# Autodesk Inventor assembly: Montagem1
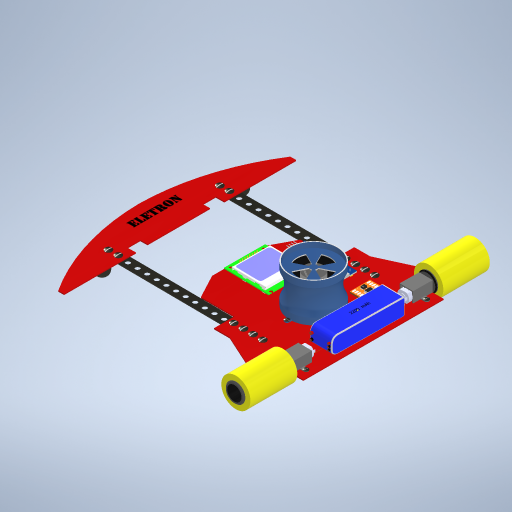
[picture p0: Inventor's stored thumbnail of the model, 512x512]
Saved by Autodesk Inventor 2023 (Build 270158000, 158)
## iProperties
Created: 2023-08-10
Part Number: Montagem1
Document SubType Name: Assembly
Designer: azeve
Author: azeve
## Documents named in this file (19)
- C:\Users\azeve\OneDrive\Área de Trabalho\seguidor_linha\Montagem1.iam
- C:\Users\azeve\OneDrive\Área de Trabalho\seguidor_linha\base_1.ipt
- C:\Users\azeve\OneDrive\Área de Trabalho\seguidor_linha\roda.ipt
- C:\Users\azeve\OneDrive\Área de Trabalho\cad_seguidor\Peças GrabCad\n20-motor-1.snapshot.1\N20 Motor.ipt
- C:\Users\azeve\OneDrive\Área de Trabalho\seguidor_linha\engate_motor.ipt
- C:\Users\azeve\OneDrive\Área de Trabalho\seguidor_linha\bateria.ipt
- C:\Users\azeve\OneDrive\Área de Trabalho\seguidor_linha\acoplamento_ventoinha1.ipt
- C:\Users\azeve\OneDrive\Área de Trabalho\seguidor_linha\aste2.ipt
- C:\Users\azeve\OneDrive\Área de Trabalho\seguidor_linha\sensor3.ipt
- C:\Users\azeve\OneDrive\Área de Trabalho\seguidor_linha\esfera.ipt
- C:\Users\azeve\OneDrive\Área de Trabalho\seguidor_linha\acoplamento_esfera.ipt
- C:\Users\azeve\OneDrive\Área de Trabalho\seguidor_linha\pneu.ipt
- C:\Users\azeve\OneDrive\Área de Trabalho\seguidor_linha\motor_ven.ipt
- C:\Users\azeve\OneDrive\Área de Trabalho\seguidor_linha\prafuso3.ipt
- C:\Users\azeve\OneDrive\Área de Trabalho\seguidor_linha\parafusos.ipt
- C:\Users\azeve\OneDrive\Área de Trabalho\seguidor_linha\helice.ipt
- C:\Users\azeve\OneDrive\Área de Trabalho\cad_seguidor\Peças GrabCad\nokia-5110-1.snapshot.1\Nokia 5110.ipt
- C:\Users\azeve\OneDrive\Área de Trabalho\cad_seguidor\Peças GrabCad\sparkfun-motor-driver-dual-tb6612fng-1a-1.snapshot.5\Motor Driver.ipt
- C:\Users\azeve\OneDrive\Área de Trabalho\cad_seguidor\Peças GrabCad\stm32f103c8t6-board-1.snapshot.2\stm32f103c8t6-board.ipt
## Components (43 placed, 18 different names)
1. base_1:1 — Coincidente:3, Coincidente:5, Coincidente:7, Coincidente:8, Coincidente:10, Coincidente:12, Alinhado:1, Inserir:20, Inserir:21, Inserir:22, Inserir:23, Inserir:24, Inserir:25, Inserir:26, Inserir:27, Coincidente:16, Coincidente:17
2. roda:1 — Inserir:4, Inserir:6
3. roda:2 — Inserir:3, Inserir:5
4. N20 Motor:1 — Coincidente:3, Coincidente:4, Inserir:4
5. N20 Motor:2 — Coincidente:1, Coincidente:2, Coincidente:5, Inserir:3
6. engate_motor:1 — Inserir:12, Inserir:13
7. engate_motor:2 — Inserir:14, Inserir:15
8. bateria:1
9. acoplamento_ventoinha1:1 — Inserir:7, Inserir:8, Inserir:9, Inserir:10, Inserir:11, Inserir:28
10. aste2:1 — Coincidente:8, Coincidente:11, Coincidente:12
11. aste2:2 — Coincidente:7, Coincidente:9, Coincidente:10
12. sensor3:1 — Coincidente:9, Coincidente:11, Coincidente:14, Coincidente:15, Inserir:16, Inserir:17, Inserir:18, Inserir:19
13. esfera:1 — Tangente:1
14. esfera:2 — Coincidente:13
15. acoplamento_esfera:1 — Tangente:1, Coincidente:15
16. acoplamento_esfera:2 — Coincidente:13, Coincidente:14
17. pneu:1 — Inserir:5
18. pneu:2 — Inserir:6
19. motor_ven:1 — Inserir:7
20. prafuso3:1 — Inserir:9
21. prafuso3:2 — Inserir:15
22. prafuso3:3 — Inserir:11
23. prafuso3:4 — Inserir:8
24. prafuso3:5 — Inserir:13
25. prafuso3:6 — Inserir:12
26. prafuso3:7 — Inserir:14
27. prafuso3:8 — Inserir:10
28. parafusos:1 — Inserir:20
29. parafusos:2 — Inserir:21
30. parafusos:3 — Inserir:22
31. parafusos:4 — Inserir:23
32. parafusos:5 — Inserir:24
33. parafusos:6 — Inserir:27
34. parafusos:7 — Inserir:25
35. parafusos:8 — Inserir:26
36. parafusos:9 — Inserir:18
37. parafusos:10 — Inserir:19
38. parafusos:11 — Inserir:16
39. parafusos:12 — Inserir:17
40. helice:1 — Inserir:28
41. Nokia 5110:1
42. Motor Driver:1 — Coincidente:16
43. stm32f103c8t6-board:1 — Coincidente:17
## Relationships (45: Insert 26, Mate 16, Flush 2, Tangent 1)
- Coincidente:1 [Mate]: N20 Motor:2
- Coincidente:2 [Mate]: N20 Motor:2
- Coincidente:3 [Mate]: base_1:1 ↔ N20 Motor:1
- Coincidente:4 [Mate]: N20 Motor:1
- Coincidente:5 [Mate]: base_1:1 ↔ N20 Motor:2
- Inserir:3: roda:2 ↔ N20 Motor:2
- Inserir:4: roda:1 ↔ N20 Motor:1
- Coincidente:7 [Mate]: base_1:1 ↔ aste2:2
- Coincidente:8 [Mate]: base_1:1 ↔ aste2:1
- Coincidente:9 [Mate]: aste2:2 ↔ sensor3:1
- Coincidente:10 [Mate]: base_1:1 ↔ aste2:2
- Coincidente:11 [Mate]: aste2:1 ↔ sensor3:1
- Coincidente:12 [Mate]: base_1:1 ↔ aste2:1
- Tangente:1: esfera:1 ↔ acoplamento_esfera:1
- Coincidente:13 [Mate]: esfera:2 ↔ acoplamento_esfera:2
- Coincidente:14 [Mate]: sensor3:1 ↔ acoplamento_esfera:2
- Coincidente:15 [Mate]: sensor3:1 ↔ acoplamento_esfera:1
- Inserir:5: roda:2 ↔ pneu:1
- Inserir:6: roda:1 ↔ pneu:2
- Alinhado:1 [Flush]: base_1:1
- Alinhado:2 [Flush] (3.5 mm)
- Inserir:7: acoplamento_ventoinha1:1 ↔ motor_ven:1
- Inserir:8: acoplamento_ventoinha1:1 ↔ prafuso3:4
- Inserir:9: acoplamento_ventoinha1:1 ↔ prafuso3:1
- Inserir:10: acoplamento_ventoinha1:1 ↔ prafuso3:8
- Inserir:11: acoplamento_ventoinha1:1 ↔ prafuso3:3
- Inserir:12: engate_motor:1 ↔ prafuso3:6
- Inserir:13: engate_motor:1 ↔ prafuso3:5
- Inserir:14: engate_motor:2 ↔ prafuso3:7
- Inserir:15: engate_motor:2 ↔ prafuso3:2
- Inserir:16: sensor3:1 ↔ parafusos:11
- Inserir:17: sensor3:1 ↔ parafusos:12
- Inserir:18: sensor3:1 ↔ parafusos:9
- Inserir:19: sensor3:1 ↔ parafusos:10
- Inserir:20: base_1:1 ↔ parafusos:1
- Inserir:21: base_1:1 ↔ parafusos:2
- Inserir:22: base_1:1 ↔ parafusos:3
- Inserir:23: base_1:1 ↔ parafusos:4
- Inserir:24: base_1:1 ↔ parafusos:5
- Inserir:25: base_1:1 ↔ parafusos:7
- Inserir:26: base_1:1 ↔ parafusos:8
- Inserir:27: base_1:1 ↔ parafusos:6
- Inserir:28: acoplamento_ventoinha1:1 ↔ helice:1
- Coincidente:16 [Mate]: base_1:1 ↔ Motor Driver:1
- Coincidente:17 [Mate]: base_1:1 ↔ stm32f103c8t6-board:1
